# Autodesk Inventor assembly: gantry_assembly
(part 2 of 2)
- Slider:43 [TranslationJoint]: makerbeam876mm:2 ↔ M3_Lock_Nut(Thin_Nut):43
- Slider:44 [TranslationJoint]: makerbeam876mm:2 ↔ M3_Lock_Nut(Thin_Nut):46
- Slider:45 [TranslationJoint]: makerbeam876mm:2 ↔ M3_Lock_Nut(Thin_Nut):47
- Slider:46 [TranslationJoint]: makerbeam876mm:2 ↔ M3_Lock_Nut(Thin_Nut):48
- Slider:47 [TranslationJoint]: makerbeam876mm:4 ↔ M3_Lock_Nut(Thin_Nut):49
- Slider:48 [TranslationJoint]: makerbeam876mm:4 ↔ M3_Lock_Nut(Thin_Nut):50
- Flush:60 (5 mm): tieplate_small:7 ↔ M3_Lock_Nut(Thin_Nut):49
- Flush:61 (5 mm): tieplate_small:9 ↔ M3_Lock_Nut(Thin_Nut):47
- Flush:62 (5 mm): tieplate_small:6 ↔ M3_Lock_Nut(Thin_Nut):46
- Flush:63 (5 mm): tieplate_small:8 ↔ M3_Lock_Nut(Thin_Nut):45
- Mate:100 (-10.5 mm): tieplate_small:7 ↔ M3_Lock_Nut(Thin_Nut):50
- Mate:101 (-10.5 mm): tieplate_small:8 ↔ M3_Lock_Nut(Thin_Nut):44
- Mate:102 (-10.5 mm): tieplate_small:9 ↔ M3_Lock_Nut(Thin_Nut):48
- Mate:103 (-10.5 mm): tieplate_small:6 ↔ M3_Lock_Nut(Thin_Nut):43
- Cylindrical:43: M3_Lock_Nut(Thin_Nut):50 ↔ M3 X 10mm Screw:50
- Cylindrical:44: M3_Lock_Nut(Thin_Nut):49 ↔ M3 X 10mm Screw:51
- Cylindrical:45: M3_Lock_Nut(Thin_Nut):47 ↔ M3 X 10mm Screw:52
- Cylindrical:46: M3_Lock_Nut(Thin_Nut):48 ↔ M3 X 10mm Screw:49
- Cylindrical:47: M3_Lock_Nut(Thin_Nut):44 ↔ M3 X 10mm Screw:44
- Cylindrical:48: M3_Lock_Nut(Thin_Nut):45 ↔ M3 X 10mm Screw:42
- Cylindrical:49: M3_Lock_Nut(Thin_Nut):43 ↔ M3 X 10mm Screw:41
- Cylindrical:50: M3_Lock_Nut(Thin_Nut):46 ↔ M3 X 10mm Screw:43
- Mate:104: tieplate_small:6 ↔ M3 X 10mm Screw:41
- Mate:105: tieplate_small:6 ↔ M3 X 10mm Screw:43
- Mate:106: tieplate_small:8 ↔ M3 X 10mm Screw:44
- Mate:107: tieplate_small:8 ↔ M3 X 10mm Screw:42
- Mate:108: tieplate_small:7 ↔ M3 X 10mm Screw:51
- Mate:109: tieplate_small:7 ↔ M3 X 10mm Screw:50
- Mate:110: tieplate_small:9 ↔ M3 X 10mm Screw:49
- Mate:111: tieplate_small:9 ↔ M3 X 10mm Screw:52
- Slider:49 [TranslationJoint]: makerbeam876mm:3 ↔ M3_Lock_Nut(Thin_Nut):53
- Slider:50 [TranslationJoint]: makerbeam876mm:3 ↔ M3_Lock_Nut(Thin_Nut):51
- Slider:51 [TranslationJoint]: makerbeam876mm:1 ↔ M3_Lock_Nut(Thin_Nut):54
- Slider:52 [TranslationJoint]: makerbeam876mm:1 ↔ M3_Lock_Nut(Thin_Nut):52
- Flush:64 (5 mm): tieplate_small:6 ↔ M3_Lock_Nut(Thin_Nut):54
- Flush:65 (5 mm): tieplate_small:6 ↔ M3_Lock_Nut(Thin_Nut):52
- Flush:66 (5 mm): tieplate_small:7 ↔ M3_Lock_Nut(Thin_Nut):51
- Mate:112 (-10.5 mm): tieplate_small:7 ↔ M3_Lock_Nut(Thin_Nut):53
- Cylindrical:51: M3_Lock_Nut(Thin_Nut):51 ↔ M3 X 10mm Screw:46
- Cylindrical:52: M3_Lock_Nut(Thin_Nut):53 ↔ M3 X 10mm Screw:48
- Cylindrical:53: M3_Lock_Nut(Thin_Nut):54 ↔ M3 X 10mm Screw:45
- Cylindrical:54: M3_Lock_Nut(Thin_Nut):52 ↔ M3 X 10mm Screw:47
- Mate:113: tieplate_small:6 ↔ M3 X 10mm Screw:47
- Mate:114: tieplate_small:6 ↔ M3 X 10mm Screw:45
- Mate:115: tieplate_small:7 ↔ M3 X 10mm Screw:46
- Mate:116: tieplate_small:7 ↔ M3 X 10mm Screw:50
- Mate:117: tieplate_small:7 ↔ M3 X 10mm Screw:48
- Flush:67: tieplate_small:5 ↔ makerbeam876mm:4
- Flush:68: tieplate_small_MIR2:1 ↔ makerbeam876mm:4
- Flush:69: tieplate_small_MIR2:1 ↔ makerbeam876mm:2
- Flush:70: tieplate_small:5 ↔ makerbeam876mm:2
- Symmetry:1: makerbeam876mm:3 ↔ makerbeam876mm:4
- Flush:73 (300 mm): makerbeam600mm_MIR:2 ↔ tieplate_small_MIR3:1
- Mate:118: makerbeam600mm_MIR:1 ↔ tieplate_small_MIR3:1
- Mate:119: makerbeam600mm_MIR:2 ↔ tieplate_small_MIR3:1
- Flush:74 (300 mm): makerbeam600mm_MIR:4 ↔ tieplate_small_MIR3:2
- Mate:120: makerbeam600mm_MIR:4 ↔ tieplate_small_MIR3:2
- Mate:121: makerbeam600mm_MIR:3 ↔ tieplate_small_MIR3:2
- Mate:122: tieplate_small_MIR3:1 ↔ tieplate_small_MIR3:3
- Mate:123: tieplate_small_MIR3:2 ↔ tieplate_small_MIR3:3
- Mate:124: makerbeam600mm_MIR:4 ↔ tieplate_small_MIR3:3
- Flush:75: makerbeam600mm_MIR:1 ↔ tieplate_small_MIR3:3
- Flush:76: makerbeam600mm_MIR:1 ↔ tieplate_small_MIR3:3
- Mate:125: makerbeam600mm_MIR:1 ↔ tieplate_small_MIR3:3
- Flush:77: makerbeam600mm_MIR:4 ↔ tieplate_small_MIR3:3
- Flush:78: makerbeam600mm_MIR:4 ↔ tieplate_small_MIR3:3
- Flush:79 (-72.5 mm): makerbeam600mm_MIR:1 ↔ tieplate_small_MIR3:4
- Flush:80: makerbeam600mm_MIR:1 ↔ tieplate_small_MIR3:4
- Mate:126: makerbeam600mm_MIR:2 ↔ tieplate_small_MIR3:4
- Flush:81 (-72.5 mm): makerbeam600mm_MIR:3 ↔ tieplate_small_MIR3:5
- Mate:127: makerbeam600mm_MIR:4 ↔ tieplate_small_MIR3:5
- Flush:82 (10 mm): makerbeam600mm_MIR:4 ↔ tieplate_small_MIR3:6
- Mate:128: tieplate_small_MIR3:3 ↔ tieplate_small_MIR3:6
- Flush:83 (-10 mm): makerbeam600mm_MIR:3 ↔ tieplate_small_MIR3:6
- Flush:84: makerbeam600mm_MIR:4 ↔ tieplate_small_MIR3:6
- Mate:129: makerbeam600mm_MIR:3 ↔ tieplate_small_MIR3:6
- Mate:130: tieplate_small_MIR3:3 ↔ tieplate_small_MIR3:7
- Flush:85 (-10 mm): makerbeam600mm_MIR:2 ↔ tieplate_small_MIR3:7
- Flush:86: makerbeam600mm_MIR:2 ↔ tieplate_small_MIR3:7
- Mate:131: makerbeam600mm_MIR:1 ↔ tieplate_small_MIR3:7
- Flush:87 (-50 mm): makerbeam600mm_MIR:4 ↔ tieplate_big_MIR:1
- Mate:132 (-70 mm): makerbeam600mm_MIR:2 ↔ tieplate_big_MIR:1
- Mate:133: makerbeam600mm_MIR:2 ↔ tieplate_big_MIR:1
- Mate:134: tieplate_small_MIR3:3 ↔ M3 X 10mm Screw_MIR5:4
- Mate:135: tieplate_small_MIR3:3 ↔ M3 X 10mm Screw_MIR5:5
- Mate:136: tieplate_small_MIR3:3 ↔ M3 X 10mm Screw_MIR5:6
- Mate:137: tieplate_small_MIR3:3 ↔ M3 X 10mm Screw_MIR5:7
- Mate:138: tieplate_small_MIR3:5 ↔ M3 X 10mm Screw_MIR5:9
- Mate:139: tieplate_small_MIR3:4 ↔ M3 X 10mm Screw_MIR5:10
- Mate:140: tieplate_small_MIR3:5 ↔ M3 X 10mm Screw_MIR5:11
- Mate:141: tieplate_small_MIR3:3 ↔ M3 X 10mm Screw_MIR5:13
- Mate:142: tieplate_small_MIR3:3 ↔ M3 X 10mm Screw_MIR5:14
- Flush:88 (62.5 mm): tieplate_small_MIR3:6 ↔ M3_Lock_Nut(Thin_Nut)_MIR8:1
- Flush:89 (62.5 mm): tieplate_small_MIR3:6 ↔ M3_Lock_Nut(Thin_Nut)_MIR8:2
- Flush:90 (62.5 mm): tieplate_small_MIR3:7 ↔ M3_Lock_Nut(Thin_Nut)_MIR8:3
- Flush:91 (62.5 mm): makerbeam600mm_MIR:1 ↔ M3_Lock_Nut(Thin_Nut)_MIR8:4
- Mate:143 (-10.5 mm): tieplate_small_MIR3:3 ↔ M3_Lock_Nut(Thin_Nut)_MIR8:5
- Mate:144 (-10.5 mm): tieplate_small_MIR3:4 ↔ M3_Lock_Nut(Thin_Nut)_MIR8:6
- Flush:92 (68 mm): tieplate_small_MIR3:7 ↔ M3_Lock_Nut(Thin_Nut)_MIR8:7
- Flush:93: M3_Lock_Nut(Thin_Nut)_MIR8:5 ↔ M3_Lock_Nut(Thin_Nut)_MIR8:8
- Flush:94: M3_Lock_Nut(Thin_Nut)_MIR8:4 ↔ M3_Lock_Nut(Thin_Nut)_MIR8:9
- Mate:145 (-10.5 mm): tieplate_small_MIR3:7 ↔ M3_Lock_Nut(Thin_Nut)_MIR8:10
- Mate:146 (-10.5 mm): tieplate_small_MIR3:4 ↔ M3_Lock_Nut(Thin_Nut)_MIR8:11
- Flush:95 (5 mm): makerbeam600mm_MIR:1 ↔ M3_Lock_Nut(Thin_Nut)_MIR8:12
- Flush:96: M3_Lock_Nut(Thin_Nut)_MIR8:12 ↔ M3_Lock_Nut(Thin_Nut)_MIR8:13
- Mate:147 (-10.5 mm): tieplate_small_MIR3:5 ↔ M3_Lock_Nut(Thin_Nut)_MIR8:14
- Mate:148 (-10.5 mm): tieplate_small_MIR3:5 ↔ M3_Lock_Nut(Thin_Nut)_MIR8:15
- Mate:149: tieplate_small_MIR3:3
- Mate:150: tieplate_small_MIR3:3
- Mate:151: tieplate_small_MIR3:7 ↔ tieplate_small_MIR2_MIR:1
- Mate:152: tieplate_small_MIR3:6 ↔ tieplate_small_MIR2_MIR:1
- Mate:153: M3 X 10mm Screw_MIR5:12 ↔ tieplate_small_MIR2_MIR:1
- Mate:154: M3 X 10mm Screw_MIR5:3 ↔ tieplate_small_MIR2_MIR:1
- Mate:155: M3 X 10mm Screw_MIR5:8 ↔ tieplate_small_MIR2_MIR:1
- Mate:156: M3 X 10mm Screw_MIR5:15 ↔ tieplate_small_MIR2_MIR:1
- Mate:157: M3 X 10mm Screw_MIR5:2 ↔ tieplate_small_MIR2_MIR:1
- Mate:158: M3 X 10mm Screw_MIR5:1 ↔ tieplate_small_MIR2_MIR:1
- Mate:159: makerbeam600mm_MIR:3 ↔ tieplate_small_MIR2_MIR:1
- Mate:160: makerbeam600mm_MIR:2 ↔ tieplate_small_MIR2_MIR:1
- Flush:97: makerbeam600mm_MIR:2 ↔ tieplate_small_MIR2_MIR:1
- Flush:98: makerbeam600mm_MIR:2 ↔ tieplate_small_MIR2_MIR:1
- Flush:99: makerbeam600mm_MIR:3 ↔ tieplate_small_MIR2_MIR:1
- Mate:161: tieplate_small_MIR3:4 ↔ tieplate_small_MIR2_MIR:1
- Mate:162: tieplate_small_MIR3:6 ↔ tieplate_small_MIR2_MIR:1
- Mate:163: tieplate_small_MIR2_MIR:1
- Mate:164: tieplate_small_MIR2_MIR:1
- Flush:100 (5 mm): tieplate_small_MIR2_MIR:1 ↔ M3_Lock_Nut(Thin_Nut)_MIR8:16
- Flush:101 (62.5 mm): makerbeam600mm_MIR:2 ↔ M3_Lock_Nut(Thin_Nut)_MIR8:17
- Mate:165 (-10.5 mm): tieplate_small_MIR2_MIR:1 ↔ M3_Lock_Nut(Thin_Nut)_MIR8:18
- Flush:102 (62.5 mm): tieplate_small_MIR2_MIR:1 ↔ M3_Lock_Nut(Thin_Nut)_MIR8:19
- Mate:166 (-10 mm): tieplate_small_MIR2_MIR:1 ↔ M3_Lock_Nut(Thin_Nut)_MIR8:20
- Flush:103 (5 mm): makerbeam600mm_MIR:2 ↔ M3_Lock_Nut(Thin_Nut)_MIR8:21
- Mate:167: tieplate_small_MIR3:4 ↔ M3 X 10mm Screw_MIR5:16
- Mate:168 (-10.5 mm): tieplate_small_MIR3:6 ↔ M3_Lock_Nut(Thin_Nut)_MIR8:22
- Mate:169 (-10.5 mm): tieplate_small_MIR3:6 ↔ M3_Lock_Nut(Thin_Nut)_MIR8:23
- Mate:170 (-10.5 mm): tieplate_small_MIR3:7 ↔ M3_Lock_Nut(Thin_Nut)_MIR8:24
- Mate:171: tieplate_small_MIR3:7 ↔ M3 X 10mm Screw_MIR5:17
- Mate:172: tieplate_small_MIR3:7 ↔ M3 X 10mm Screw_MIR5:18
- Mate:173: tieplate_small_MIR3:6 ↔ M3 X 10mm Screw_MIR5:19
- Mate:174: tieplate_small_MIR3:6 ↔ M3 X 10mm Screw_MIR5:20
- Mate:175: tieplate_small_MIR3:6 ↔ M3 X 10mm Screw_MIR5:21
- Mate:176: tieplate_small_MIR3:6 ↔ M3 X 10mm Screw_MIR5:22
- Mate:177: tieplate_small_MIR3:7 ↔ M3 X 10mm Screw_MIR5:23
- Mate:178: tieplate_small_MIR3:7 ↔ M3 X 10mm Screw_MIR5:24
- Mate:179: tieplate_small_MIR3:1 ↔ M3 X 10mm Screw_MIR5:25
- Mate:180: tieplate_small_MIR3:1 ↔ M3 X 10mm Screw_MIR5:26
- Mate:181: tieplate_small_MIR3:2 ↔ M3 X 10mm Screw_MIR5:27
- Mate:182: tieplate_small_MIR3:1 ↔ M3 X 10mm Screw_MIR5:28
- Mate:183: tieplate_small_MIR3:1 ↔ M3 X 10mm Screw_MIR5:29
- Mate:184: tieplate_small_MIR3:2 ↔ M3 X 10mm Screw_MIR5:30
- Mate:185: tieplate_small_MIR3:1 ↔ M3 X 10mm Screw_MIR5:31
- Mate:186: tieplate_small_MIR3:2 ↔ M3 X 10mm Screw_MIR5:32
- Mate:187: tieplate_small_MIR3:2 ↔ M3 X 10mm Screw_MIR5:33
- Mate:188: tieplate_small_MIR3:1 ↔ M3 X 10mm Screw_MIR5:34
- Mate:189: tieplate_small_MIR3:2 ↔ M3 X 10mm Screw_MIR5:35
- Mate:190: tieplate_small_MIR3:2 ↔ M3 X 10mm Screw_MIR5:36
- Flush:104 (5 mm): tieplate_small_MIR3:1 ↔ M3_Lock_Nut(Thin_Nut)_MIR8:25
- Flush:105 (120 mm): tieplate_small_MIR3:1 ↔ M3_Lock_Nut(Thin_Nut)_MIR8:26
- Flush:106 (62.5 mm): tieplate_small_MIR3:1 ↔ M3_Lock_Nut(Thin_Nut)_MIR8:27
- Flush:107 (62.5 mm): tieplate_small_MIR3:1 ↔ M3_Lock_Nut(Thin_Nut)_MIR8:28
- Flush:108 (120 mm): tieplate_small_MIR3:2 ↔ M3_Lock_Nut(Thin_Nut)_MIR8:29
- Flush:109 (120 mm): tieplate_small_MIR3:2 ↔ M3_Lock_Nut(Thin_Nut)_MIR8:30
- Flush:110 (5 mm): tieplate_small_MIR3:1 ↔ M3_Lock_Nut(Thin_Nut)_MIR8:31
- Flush:111 (5 mm): tieplate_small_MIR3:2 ↔ M3_Lock_Nut(Thin_Nut)_MIR8:32
- Flush:112 (62.5 mm): tieplate_small_MIR3:2 ↔ M3_Lock_Nut(Thin_Nut)_MIR8:33
- Flush:113 (120 mm): tieplate_small_MIR3:1 ↔ M3_Lock_Nut(Thin_Nut)_MIR8:34
- Flush:114 (62.5 mm): tieplate_small_MIR3:2 ↔ M3_Lock_Nut(Thin_Nut)_MIR8:35
- Flush:115 (5 mm): tieplate_small_MIR3:2 ↔ M3_Lock_Nut(Thin_Nut)_MIR8:36
- Mate:191 (-10.5 mm): tieplate_big_MIR:1 ↔ M3_Lock_Nut(Thin_Nut)_MIR8:37
- Mate:192 (-60.5 mm): tieplate_big_MIR:1 ↔ M3_Lock_Nut(Thin_Nut)_MIR8:38
- Mate:193 (-10.5 mm): tieplate_big_MIR:1 ↔ M3_Lock_Nut(Thin_Nut)_MIR8:39
- Mate:194 (-60.5 mm): tieplate_big_MIR:1 ↔ M3_Lock_Nut(Thin_Nut)_MIR8:40
- Mate:195: tieplate_big_MIR:1 ↔ M3 X 10mm Screw_MIR5:37
- Mate:196: tieplate_big_MIR:1 ↔ M3 X 10mm Screw_MIR5:38
- Mate:197: tieplate_big_MIR:1 ↔ M3 X 10mm Screw_MIR5:39
- Mate:198: tieplate_big_MIR:1 ↔ M3 X 10mm Screw_MIR5:40
- Mate:199 (-10.5 mm): tieplate_small_MIR3:4 ↔ M3_Lock_Nut(Thin_Nut)_MIR8:41
- Mate:200 (-10.5 mm): tieplate_small_MIR3:6 ↔ M3_Lock_Nut(Thin_Nut)_MIR8:42
- Flush:116 (5 mm): tieplate_small_MIR3:6 ↔ M3_Lock_Nut(Thin_Nut)_MIR8:43
- Flush:117 (5 mm): tieplate_small_MIR3:4 ↔ M3_Lock_Nut(Thin_Nut)_MIR8:44
- Flush:118 (5 mm): tieplate_small_MIR3:7 ↔ M3_Lock_Nut(Thin_Nut)_MIR8:45
- Mate:201 (-10.5 mm): tieplate_small_MIR3:7 ↔ M3_Lock_Nut(Thin_Nut)_MIR8:46
- Flush:119 (5 mm): tieplate_small_MIR3:5 ↔ M3_Lock_Nut(Thin_Nut)_MIR8:47
- Mate:202 (-10.5 mm): tieplate_small_MIR3:5 ↔ M3_Lock_Nut(Thin_Nut)_MIR8:48
- Flush:121 (5 mm): tieplate_small_MIR3:4 ↔ M3_Lock_Nut(Thin_Nut)_MIR8:50
- Mate:204: tieplate_small_MIR3:4 ↔ M3 X 10mm Screw_MIR5:41
- Mate:205: tieplate_small_MIR3:6 ↔ M3 X 10mm Screw_MIR5:42
- Mate:206: tieplate_small_MIR3:4 ↔ M3 X 10mm Screw_MIR5:43
- Mate:207: tieplate_small_MIR3:6 ↔ M3 X 10mm Screw_MIR5:44
- Mate:209: tieplate_small_MIR3:5 ↔ M3 X 10mm Screw_MIR5:46
- Mate:210: tieplate_small_MIR3:4 ↔ M3 X 10mm Screw_MIR5:47
- Mate:211: tieplate_small_MIR3:5 ↔ M3 X 10mm Screw_MIR5:48
- Mate:212: tieplate_small_MIR3:7 ↔ M3 X 10mm Screw_MIR5:49
- Mate:213: tieplate_small_MIR3:5 ↔ M3 X 10mm Screw_MIR5:50
- Mate:214: tieplate_small_MIR3:5 ↔ M3 X 10mm Screw_MIR5:50
- Mate:215: tieplate_small_MIR3:5 ↔ M3 X 10mm Screw_MIR5:51
- Mate:216: tieplate_small_MIR3:7 ↔ M3 X 10mm Screw_MIR5:52
- Slider:53 [TranslationJoint]: makerbeam600mm_MIR:4 ↔ M3_Lock_Nut(Thin_Nut)_MIR8:1
- Slider:54 [TranslationJoint]: makerbeam600mm_MIR:3 ↔ M3_Lock_Nut(Thin_Nut)_MIR8:2
- Slider:55 [TranslationJoint]: makerbeam600mm_MIR:1 ↔ M3_Lock_Nut(Thin_Nut)_MIR8:3
- Cylindrical:55: M3 X 10mm Screw_MIR5:4 ↔ M3_Lock_Nut(Thin_Nut)_MIR8:4
- Slider:56 [TranslationJoint]: makerbeam600mm_MIR:1 ↔ M3_Lock_Nut(Thin_Nut)_MIR8:4
- Cylindrical:56: M3 X 10mm Screw_MIR5:14 ↔ M3_Lock_Nut(Thin_Nut)_MIR8:5
- Slider:57 [TranslationJoint]: makerbeam600mm_MIR:1 ↔ M3_Lock_Nut(Thin_Nut)_MIR8:5
- Slider:58 [TranslationJoint]: makerbeam600mm_MIR:2 ↔ M3_Lock_Nut(Thin_Nut)_MIR8:6
- Slider:59 [TranslationJoint]: makerbeam600mm_MIR:2 ↔ M3_Lock_Nut(Thin_Nut)_MIR8:7
- Cylindrical:57: M3 X 10mm Screw_MIR5:7 ↔ M3_Lock_Nut(Thin_Nut)_MIR8:8
- Slider:60 [TranslationJoint]: makerbeam600mm_MIR:4 ↔ M3_Lock_Nut(Thin_Nut)_MIR8:8
- Cylindrical:58: M3 X 10mm Screw_MIR5:6 ↔ M3_Lock_Nut(Thin_Nut)_MIR8:9
- Slider:61 [TranslationJoint]: makerbeam600mm_MIR:4 ↔ M3_Lock_Nut(Thin_Nut)_MIR8:9
- Slider:62 [TranslationJoint]: makerbeam600mm_MIR:2 ↔ M3_Lock_Nut(Thin_Nut)_MIR8:10
- Cylindrical:59: M3 X 10mm Screw_MIR5:10 ↔ M3_Lock_Nut(Thin_Nut)_MIR8:11
- Slider:63 [TranslationJoint]: makerbeam600mm_MIR:1 ↔ M3_Lock_Nut(Thin_Nut)_MIR8:11
- Cylindrical:60: M3 X 10mm Screw_MIR5:5 ↔ M3_Lock_Nut(Thin_Nut)_MIR8:12
- Slider:64 [TranslationJoint]: makerbeam600mm_MIR:1 ↔ M3_Lock_Nut(Thin_Nut)_MIR8:12
- Cylindrical:61: M3 X 10mm Screw_MIR5:13 ↔ M3_Lock_Nut(Thin_Nut)_MIR8:13
- Slider:65 [TranslationJoint]: makerbeam600mm_MIR:4 ↔ M3_Lock_Nut(Thin_Nut)_MIR8:13
- Cylindrical:62: M3 X 10mm Screw_MIR5:11 ↔ M3_Lock_Nut(Thin_Nut)_MIR8:14
- Slider:66 [TranslationJoint]: makerbeam600mm_MIR:4 ↔ M3_Lock_Nut(Thin_Nut)_MIR8:14
- Cylindrical:63: M3 X 10mm Screw_MIR5:9 ↔ M3_Lock_Nut(Thin_Nut)_MIR8:15
- Slider:67 [TranslationJoint]: makerbeam600mm_MIR:3 ↔ M3_Lock_Nut(Thin_Nut)_MIR8:15
- Cylindrical:64: M3 X 10mm Screw_MIR5:2 ↔ M3_Lock_Nut(Thin_Nut)_MIR8:16
- Slider:68 [TranslationJoint] (2.4 mm): makerbeam600mm_MIR:3 ↔ M3_Lock_Nut(Thin_Nut)_MIR8:16
- Cylindrical:65: M3 X 10mm Screw_MIR5:15 ↔ M3_Lock_Nut(Thin_Nut)_MIR8:17
- Slider:69 [TranslationJoint] (2.4 mm): makerbeam600mm_MIR:2 ↔ M3_Lock_Nut(Thin_Nut)_MIR8:17
- Cylindrical:66: M3 X 10mm Screw_MIR5:3 ↔ M3_Lock_Nut(Thin_Nut)_MIR8:18
- Slider:70 [TranslationJoint] (2.4 mm): makerbeam600mm_MIR:3 ↔ M3_Lock_Nut(Thin_Nut)_MIR8:18
- Cylindrical:67: M3 X 10mm Screw_MIR5:12 ↔ M3_Lock_Nut(Thin_Nut)_MIR8:19
- Slider:71 [TranslationJoint] (2.4 mm): makerbeam600mm_MIR:3 ↔ M3_Lock_Nut(Thin_Nut)_MIR8:19
- Cylindrical:68: M3 X 10mm Screw_MIR5:8 ↔ M3_Lock_Nut(Thin_Nut)_MIR8:20
- Slider:72 [TranslationJoint] (2.4 mm): makerbeam600mm_MIR:2 ↔ M3_Lock_Nut(Thin_Nut)_MIR8:20
- Cylindrical:69: M3 X 10mm Screw_MIR5:1 ↔ M3_Lock_Nut(Thin_Nut)_MIR8:21
- Slider:73 [TranslationJoint]: makerbeam600mm_MIR:2 ↔ M3_Lock_Nut(Thin_Nut)_MIR8:21
- Cylindrical:70: M3_Lock_Nut(Thin_Nut)_MIR8:6 ↔ M3 X 10mm Screw_MIR5:16
- Slider:74 [TranslationJoint]: makerbeam600mm_MIR:3 ↔ M3_Lock_Nut(Thin_Nut)_MIR8:22
- Slider:75 [TranslationJoint]: makerbeam600mm_MIR:4 ↔ M3_Lock_Nut(Thin_Nut)_MIR8:23
- Slider:76 [TranslationJoint]: makerbeam600mm_MIR:1 ↔ M3_Lock_Nut(Thin_Nut)_MIR8:24
- Cylindrical:71: M3_Lock_Nut(Thin_Nut)_MIR8:3 ↔ M3 X 10mm Screw_MIR5:17
- Cylindrical:72: M3_Lock_Nut(Thin_Nut)_MIR8:7 ↔ M3 X 10mm Screw_MIR5:18
- Cylindrical:73: M3_Lock_Nut(Thin_Nut)_MIR8:2 ↔ M3 X 10mm Screw_MIR5:19
- Cylindrical:74: M3_Lock_Nut(Thin_Nut)_MIR8:1 ↔ M3 X 10mm Screw_MIR5:20
- Cylindrical:75: M3_Lock_Nut(Thin_Nut)_MIR8:22 ↔ M3 X 10mm Screw_MIR5:21
- Cylindrical:76: M3_Lock_Nut(Thin_Nut)_MIR8:23 ↔ M3 X 10mm Screw_MIR5:22
- Cylindrical:77: M3_Lock_Nut(Thin_Nut)_MIR8:24 ↔ M3 X 10mm Screw_MIR5:23
- Cylindrical:78: M3_Lock_Nut(Thin_Nut)_MIR8:10 ↔ M3 X 10mm Screw_MIR5:24
- Cylindrical:79: M3 X 10mm Screw_MIR5:26 ↔ M3_Lock_Nut(Thin_Nut)_MIR8:25
- Slider:77 [TranslationJoint]: makerbeam600mm_MIR:2 ↔ M3_Lock_Nut(Thin_Nut)_MIR8:25
- Cylindrical:80: M3 X 10mm Screw_MIR5:31 ↔ M3_Lock_Nut(Thin_Nut)_MIR8:26
- Slider:78 [TranslationJoint]: makerbeam600mm_MIR:2 ↔ M3_Lock_Nut(Thin_Nut)_MIR8:26
- Cylindrical:81: M3 X 10mm Screw_MIR5:28 ↔ M3_Lock_Nut(Thin_Nut)_MIR8:27
- Slider:79 [TranslationJoint]: makerbeam600mm_MIR:1 ↔ M3_Lock_Nut(Thin_Nut)_MIR8:27
- Cylindrical:82: M3 X 10mm Screw_MIR5:29 ↔ M3_Lock_Nut(Thin_Nut)_MIR8:28
- Slider:80 [TranslationJoint]: makerbeam600mm_MIR:2 ↔ M3_Lock_Nut(Thin_Nut)_MIR8:28
- Cylindrical:83: M3 X 10mm Screw_MIR5:36 ↔ M3_Lock_Nut(Thin_Nut)_MIR8:29
- Slider:81 [TranslationJoint]: makerbeam600mm_MIR:4 ↔ M3_Lock_Nut(Thin_Nut)_MIR8:29
- Cylindrical:84: M3 X 10mm Screw_MIR5:32 ↔ M3_Lock_Nut(Thin_Nut)_MIR8:30
- Slider:82 [TranslationJoint]: makerbeam600mm_MIR:3 ↔ M3_Lock_Nut(Thin_Nut)_MIR8:30
- Cylindrical:85: M3 X 10mm Screw_MIR5:25 ↔ M3_Lock_Nut(Thin_Nut)_MIR8:31
- Slider:83 [TranslationJoint]: makerbeam600mm_MIR:1 ↔ M3_Lock_Nut(Thin_Nut)_MIR8:31
- Cylindrical:86: M3 X 10mm Screw_MIR5:35 ↔ M3_Lock_Nut(Thin_Nut)_MIR8:32
- Slider:84 [TranslationJoint]: makerbeam600mm_MIR:3 ↔ M3_Lock_Nut(Thin_Nut)_MIR8:32
- Cylindrical:87: M3 X 10mm Screw_MIR5:33 ↔ M3_Lock_Nut(Thin_Nut)_MIR8:33
- Slider:85 [TranslationJoint]: makerbeam600mm_MIR:4 ↔ M3_Lock_Nut(Thin_Nut)_MIR8:33
- Cylindrical:88: M3 X 10mm Screw_MIR5:34 ↔ M3_Lock_Nut(Thin_Nut)_MIR8:34
- Slider:86 [TranslationJoint]: makerbeam600mm_MIR:1 ↔ M3_Lock_Nut(Thin_Nut)_MIR8:34
- Cylindrical:89: M3 X 10mm Screw_MIR5:27 ↔ M3_Lock_Nut(Thin_Nut)_MIR8:35
- Slider:87 [TranslationJoint]: makerbeam600mm_MIR:3 ↔ M3_Lock_Nut(Thin_Nut)_MIR8:35
- Cylindrical:90: M3 X 10mm Screw_MIR5:30 ↔ M3_Lock_Nut(Thin_Nut)_MIR8:36
- Slider:88 [TranslationJoint]: makerbeam600mm_MIR:4 ↔ M3_Lock_Nut(Thin_Nut)_MIR8:36
- Slider:89 [TranslationJoint]: makerbeam600mm_MIR:3 ↔ M3_Lock_Nut(Thin_Nut)_MIR8:37
- Slider:90 [TranslationJoint]: makerbeam600mm_MIR:3 ↔ M3_Lock_Nut(Thin_Nut)_MIR8:38
- Slider:91 [TranslationJoint]: makerbeam600mm_MIR:2 ↔ M3_Lock_Nut(Thin_Nut)_MIR8:39
- Slider:92 [TranslationJoint]: makerbeam600mm_MIR:2 ↔ M3_Lock_Nut(Thin_Nut)_MIR8:40
- Cylindrical:91: M3_Lock_Nut(Thin_Nut)_MIR8:38 ↔ M3 X 10mm Screw_MIR5:37
- Cylindrical:92: M3_Lock_Nut(Thin_Nut)_MIR8:37 ↔ M3 X 10mm Screw_MIR5:38
- Cylindrical:93: M3_Lock_Nut(Thin_Nut)_MIR8:40 ↔ M3 X 10mm Screw_MIR5:39
- Cylindrical:94: M3_Lock_Nut(Thin_Nut)_MIR8:39 ↔ M3 X 10mm Screw_MIR5:40
- Cylindrical:95: M3_Lock_Nut(Thin_Nut)_MIR8:41 ↔ M3 X 10mm Screw_MIR5:41
- Cylindrical:96: M3_Lock_Nut(Thin_Nut)_MIR8:43 ↔ M3 X 10mm Screw_MIR5:42
- Cylindrical:97: M3_Lock_Nut(Thin_Nut)_MIR8:44 ↔ M3 X 10mm Screw_MIR5:43
- Cylindrical:98: M3_Lock_Nut(Thin_Nut)_MIR8:42 ↔ M3 X 10mm Screw_MIR5:44
- Cylindrical:99: M3_Lock_Nut(Thin_Nut)_MIR8:52 ↔ M3 X 10mm Screw_MIR5:45
- Cylindrical:100: M3_Lock_Nut(Thin_Nut)_MIR8:49 ↔ M3 X 10mm Screw_MIR5:46
- Cylindrical:101: M3_Lock_Nut(Thin_Nut)_MIR8:50 ↔ M3 X 10mm Screw_MIR5:47
- Cylindrical:102: M3_Lock_Nut(Thin_Nut)_MIR8:51 ↔ M3 X 10mm Screw_MIR5:48
- Cylindrical:103: M3_Lock_Nut(Thin_Nut)_MIR8:46 ↔ M3 X 10mm Screw_MIR5:49
- Cylindrical:104: M3_Lock_Nut(Thin_Nut)_MIR8:48 ↔ M3 X 10mm Screw_MIR5:50
- Cylindrical:105: M3_Lock_Nut(Thin_Nut)_MIR8:47 ↔ M3 X 10mm Screw_MIR5:51
- Cylindrical:106: M3_Lock_Nut(Thin_Nut)_MIR8:45 ↔ M3 X 10mm Screw_MIR5:52
- Flush:123: makerbeam876mm:4 ↔ tieplate_small_MIR3:3
- Flush:124: makerbeam876mm:4 ↔ tieplate_small_MIR2_MIR:1
- Flush:125: tieplate_small:5 ↔ makerbeam876mm:2
- Flush:126: tieplate_small_MIR2:1 ↔ makerbeam876mm:2
- Flush:127: makerbeam600mm:1 ↔ tieplate_small:5
- Flush:128: makerbeam600mm:2 ↔ tieplate_small_MIR2:1
- Flush:129: makerbeam600mm:4 ↔ tieplate_small:5
- Flush:130: makerbeam600mm:3 ↔ tieplate_small_MIR2:1
- Flush:131: makerbeam600mm:4 ↔ tieplate_small:7
- Flush:132: makerbeam600mm:1 ↔ tieplate_small:6
- Flush:133: makerbeam600mm:2 ↔ tieplate_small:6
- Flush:134: makerbeam600mm:3 ↔ tieplate_small:7
- Flush:135: tieplate_small:7 ↔ makerbeam876mm:3
- Flush:136: tieplate_small:6 ↔ makerbeam876mm:1
- Flush:137: tieplate_small:9 ↔ makerbeam876mm:2
- Flush:138: tieplate_small:8 ↔ makerbeam876mm:4
- Flush:139: makerbeam876mm:3 ↔ tieplate_small_MIR3:5
- Flush:140: makerbeam876mm:1 ↔ tieplate_small_MIR3:4
- Flush:141: makerbeam876mm:2 ↔ tieplate_small_MIR3:7
- Flush:142: makerbeam876mm:4 ↔ tieplate_small_MIR3:6
- Flush:143: makerbeam600mm_MIR:4 ↔ tieplate_small_MIR3:3
- Flush:144: makerbeam600mm_MIR:4 ↔ tieplate_small_MIR3:5
- Flush:145: makerbeam600mm_MIR:3 ↔ tieplate_small_MIR2_MIR:1
- Flush:146: makerbeam600mm_MIR:3 ↔ tieplate_small_MIR3:5
- Flush:147: makerbeam600mm:1 ↔ tieplate_small:5
- Flush:148: makerbeam600mm:1 ↔ tieplate_small:6
- Flush:149: makerbeam600mm:2 ↔ tieplate_small_MIR2:1
- Flush:150: makerbeam600mm:2 ↔ tieplate_small:6
- Flush:151: makerbeam600mm:3 ↔ tieplate_small_MIR2:1
- Flush:152: makerbeam600mm:3 ↔ tieplate_small:7
- Slider:93 [TranslationJoint]: makerbeam876mm:2 ↔ M3_Lock_Nut(Thin_Nut)_MIR8:44
- Slider:94 [TranslationJoint]: makerbeam876mm:2 ↔ M3_Lock_Nut(Thin_Nut)_MIR8:41
- Slider:95 [TranslationJoint]: makerbeam876mm:1 ↔ M3_Lock_Nut(Thin_Nut)_MIR8:50
- Slider:97 [TranslationJoint]: makerbeam876mm:4 ↔ M3_Lock_Nut(Thin_Nut)_MIR8:47
- Slider:98 [TranslationJoint]: makerbeam876mm:4 ↔ M3_Lock_Nut(Thin_Nut)_MIR8:48
- Slider:99 [TranslationJoint]: makerbeam876mm:3 ↔ M3_Lock_Nut(Thin_Nut)_MIR8:49
- Slider:100 [TranslationJoint]: makerbeam876mm:3 ↔ M3_Lock_Nut(Thin_Nut)_MIR8:51
- Flush:153 (5 mm): tieplate_small_MIR3:5 ↔ M3_Lock_Nut(Thin_Nut)_MIR8:51
- Mate:217 (-10.5 mm): tieplate_small_MIR3:5 ↔ M3_Lock_Nut(Thin_Nut)_MIR8:49
- Flush:154 (5 mm): tieplate_small_MIR3:5 ↔ M3_Lock_Nut(Thin_Nut)_MIR8:47
- Slider:101 [TranslationJoint]: makerbeam876mm:1 ↔ M3_Lock_Nut(Thin_Nut)_MIR8:52
- Flush:155 (5 mm): tieplate_small_MIR3:4 ↔ M3_Lock_Nut(Thin_Nut)_MIR8:52
- Mate:218: tieplate_small_MIR3:4 ↔ M3 X 10mm Screw_MIR5:45
- Mate:219: tieplate_small_MIR3:4 ↔ M3 X 10mm Screw_MIR5:47
- Mate:220: tieplate_small_MIR3:5 ↔ M3 X 10mm Screw_MIR5:48
- Mate:221: tieplate_small_MIR3:5 ↔ M3 X 10mm Screw_MIR5:46
- Mate:222: tieplate_small_MIR3:5 ↔ M3 X 10mm Screw_MIR5:51
- Mate:223: tieplate_small_MIR3:5 ↔ M3 X 10mm Screw_MIR5:50
- Mate:224: tieplate_small_MIR3:4 ↔ M3 X 10mm Screw_MIR5:41
- Mate:225: tieplate_small_MIR3:4 ↔ M3 X 10mm Screw_MIR5:43
- Slider:102 [TranslationJoint]: makerbeam876mm:4 ↔ M3_Lock_Nut(Thin_Nut)_MIR8:43
- Slider:103 [TranslationJoint]: makerbeam876mm:4 ↔ M3_Lock_Nut(Thin_Nut)_MIR8:42
- Slider:104 [TranslationJoint]: makerbeam876mm:2 ↔ M3_Lock_Nut(Thin_Nut)_MIR8:46
- Slider:105 [TranslationJoint]: makerbeam876mm:2 ↔ M3_Lock_Nut(Thin_Nut)_MIR8:45
- Flush:160 (-52.0465 mm): makerbeam876mm:4 ↔ tieplate_small_MIR3:5
- Symmetry:2: tieplate_small:5 ↔ tieplate_small_MIR3:3
- Mate:226 (0.1 mm): tieplate_big:1 ↔ NEMA17 w connector metric:3
- Flush:161 (50 mm): tieplate_big:1 ↔ NEMA17 w connector metric:3
- Flush:162 (20 mm): tieplate_big:1 ↔ NEMA17 w connector metric:3
- Mate:227: tieplate_big:1 ↔ M5 x 12mm Screw:1
- Flush:163 (80 mm): tieplate_big:1 ↔ M5 x 12mm Screw:1
- Mate:228 (-95 mm): tieplate_big:1 ↔ M5 x 12mm Screw:1
- Mate:229: NEMA17 w connector metric:3
- Mate:230: NEMA17 w connector metric:3
- Mate:231: NEMA17 w connector metric:3
- Flush:164 (15 mm): tieplate_big:1 ↔ M5 x 12mm Screw_MIR:1
- Mate:232: tieplate_big:1 ↔ M5 x 12mm Screw_MIR:1
- Mate:233 (-95 mm): tieplate_big:1 ↔ M5 x 12mm Screw_MIR:1
- Rigid:2 [WeldJoint]: GT2Bearing metric:4 ↔ M5 x 12mm Screw:1
- Rigid:3 [WeldJoint]: NEMA17 w connector metric:3 ↔ GT2Pulley metric:1
- Rigid:4 [WeldJoint]: GT2Bearing metric:3 ↔ M5 x 12mm Screw_MIR:1
- Mate:239: tieplate_big:1
- Mate:240: tieplate_big:1
- Mate:241: tieplate_big:1
- Mate:244: tieplate_big:1 ↔ m5x12mmscrew:1
- Cylindrical:107: tieplate_big:1 ↔ m5x12mmscrew:1
- Mate:245: tieplate_big:1 ↔ m5x12mmscrew:2
- Mate:246: tieplate_big:1 ↔ m5x12mmscrew:3
- Cylindrical:108: tieplate_big:1 ↔ m5x12mmscrew:3
- Cylindrical:109: tieplate_big:1 ↔ m5x12mmscrew:2
- Rotational:1 [RevoluteJoint] (-0.5 mm): m5x12mmscrew:2 ↔ 5mmx20mmx8mm bearing:1
- Rotational:2 [RevoluteJoint] (-0.5 mm): m5x12mmscrew:1 ↔ 5mmx20mmx8mm bearing:2
- Rotational:3 [RevoluteJoint] (-0.5 mm): m5x12mmscrew:3 ↔ 5mmx20mmx8mm bearing:3
- Mate:247: NEMA17 w connector metric_MIR:1
- Mate:248: NEMA17 w connector metric_MIR:1
- Mate:249: NEMA17 w connector metric_MIR:1
- Rigid:5 [WeldJoint]: NEMA17 w connector metric_MIR:1 ↔ GT2Pulley metric_MIR:1
- Rigid:6 [WeldJoint]: GT2Bearing metric_MIR:2 ↔ M5 x 12mm Screw_MIR1:1
- Rigid:7 [WeldJoint]: GT2Bearing metric_MIR:1 ↔ M5 x 12mm Screw_MIR_MIR:1
- Rotational:4 [RevoluteJoint] (0.5 mm): m5x12mmscrew_MIR:2 ↔ 5mmx20mmx8mm bearing_MIR:1
- Rotational:5 [RevoluteJoint] (-0.5 mm): m5x12mmscrew_MIR:1 ↔ 5mmx20mmx8mm bearing_MIR:2
- Rotational:6 [RevoluteJoint] (-0.5 mm): m5x12mmscrew_MIR:3 ↔ 5mmx20mmx8mm bearing_MIR:3
- Mate:250: tieplate_big_MIR:1 ↔ m5x12mmscrew_MIR:2
- Mate:251: tieplate_big_MIR:1 ↔ m5x12mmscrew_MIR:1
- Mate:252: tieplate_big_MIR:1 ↔ NEMA17 w connector metric_MIR:1
- Mate:253: tieplate_big_MIR:1 ↔ M5 x 12mm Screw_MIR1:1
- Mate:255: tieplate_big_MIR:1 ↔ m5x12mmscrew_MIR:3
- Mate:256: tieplate_big_MIR:1 ↔ m5x12mmscrew_MIR:1
- Cylindrical:110: tieplate_big_MIR:1 ↔ m5x12mmscrew_MIR:2
- Cylindrical:111: tieplate_big_MIR:1 ↔ m5x12mmscrew_MIR:3
- Cylindrical:112: tieplate_big_MIR:1 ↔ m5x12mmscrew_MIR:1
- Mate:257 (50 mm): tieplate_big_MIR:1 ↔ NEMA17 w connector metric_MIR:1
- Flush:165 (20 mm): tieplate_big_MIR:1 ↔ NEMA17 w connector metric_MIR:1
- Mate:258: tieplate_big_MIR:1 ↔ M5 x 12mm Screw_MIR_MIR:1
- Mate:259 (-20 mm): tieplate_big_MIR:1 ↔ M5 x 12mm Screw_MIR_MIR:1
- Flush:166: M5 x 12mm Screw_MIR1:1 ↔ M5 x 12mm Screw_MIR_MIR:1
- Mate:302 (-80 mm): tieplate_big_MIR:1 ↔ M5 x 12mm Screw_MIR_MIR:1
- Mate:303 (-80 mm): tieplate_big_MIR:1 ↔ M5 x 12mm Screw_MIR1:1
- Mate:304 (-52.5 mm): tieplate_big_MIR:1 ↔ M5 x 12mm Screw_MIR1:1
- Flush:182: makerbeam876mm:3 ↔ makerbeam_L-bracket:1
- Mate:320: makerbeam876mm:3 ↔ makerbeam_L-bracket:1
- Flush:183: makerbeam876mm:3 ↔ makerbeam_L-bracket:1
- Flush:184: makerbeam876mm:3 ↔ makerbeam_L-bracket:2
- Flush:185: makerbeam876mm:3 ↔ makerbeam_L-bracket:2
- Mate:321: makerbeam876mm:3 ↔ makerbeam_L-bracket:2
- Slider:106 [TranslationJoint]: makerbeam876mm:3 ↔ M3_Lock_Nut(Thin_Nut):55
- Slider:107 [TranslationJoint]: makerbeam876mm:3 ↔ M3_Lock_Nut(Thin_Nut):56
- Flush:186 (3 mm): makerbeam876mm:3 ↔ M3_Lock_Nut(Thin_Nut):56
- Mate:322 (-10 mm): makerbeam_L-bracket:2 ↔ M3_Lock_Nut(Thin_Nut):55
- Slider:108 [TranslationJoint]: makerbeam876mm:3 ↔ M3_Lock_Nut(Thin_Nut):57
- Slider:109 [TranslationJoint]: makerbeam876mm:3 ↔ M3_Lock_Nut(Thin_Nut):58
- Flush:187 (3 mm): makerbeam_L-bracket:1 ↔ M3_Lock_Nut(Thin_Nut):58
- Mate:323 (-10.5 mm): makerbeam_L-bracket:1 ↔ M3_Lock_Nut(Thin_Nut):57
- Cylindrical:132: M3_Lock_Nut(Thin_Nut):57 ↔ M3 X 10mm Screw:61
- Cylindrical:133: M3_Lock_Nut(Thin_Nut):58 ↔ M3 X 10mm Screw:62
- Cylindrical:134: M3_Lock_Nut(Thin_Nut):56 ↔ M3 X 10mm Screw:63
- Cylindrical:135: M3_Lock_Nut(Thin_Nut):55 ↔ M3 X 10mm Screw:64
- Mate:324: makerbeam_L-bracket:2 ↔ M3 X 10mm Screw:63
- Mate:325: makerbeam_L-bracket:1 ↔ M3 X 10mm Screw:61
- Mate:326: makerbeam_L-bracket:1 ↔ M3 X 10mm Screw:62
- Mate:327: makerbeam_L-bracket:2 ↔ M3 X 10mm Screw:64
- Cylindrical:136: makerbeam_L-bracket:2 ↔ M3 X 10mm Screw:65
- Cylindrical:137: makerbeam_L-bracket:1 ↔ M3 X 10mm Screw:66
- Mate:328: makerbeam_L-bracket:1 ↔ M3 X 10mm Screw:66
- Mate:329: makerbeam_L-bracket:2 ↔ M3 X 10mm Screw:65
- Cylindrical:138: M3 X 10mm Screw:65 ↔ M3_Lock_Nut(Thin_Nut):59
- Cylindrical:139: M3 X 10mm Screw:66 ↔ M3_Lock_Nut(Thin_Nut):60
- Mate:330: makerbeam_L-bracket:1 ↔ M3_Lock_Nut(Thin_Nut):60
- Mate:331: makerbeam_L-bracket:2 ↔ M3_Lock_Nut(Thin_Nut):59
- Flush:188: makerbeam876mm:2 ↔ makerbeam876mm:4
- Flush:189: makerbeam876mm:1 ↔ makerbeam876mm:2
- Flush:190: makerbeam876mm:1 ↔ makerbeam876mm:3
- Flush:191: makerbeam876mm:3 ↔ makerbeam876mm:4
- Flush:192: makerbeam876mm:1 ↔ makerbeam876mm:4
